# Autodesk Inventor assembly: Ensamblaje
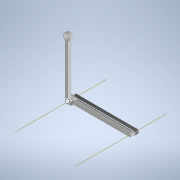
[picture p0: Inventor's stored thumbnail of the model, 180x180]
Saved by Autodesk Inventor 2021 (Build 250183000, 183)
## iProperties
Created: 2022-10-24
Part Number: Ensamblaje
Document SubType Name: Assembly
Designer: ivanm
Author: ivanm
## Documents named in this file (6)
- C:\Users\ivanm\OneDrive\Servomecanismos\Proyectos\Proyecto academico\Servomecanismo2R\INVENTOR\Ensamblaje.iam
- C:\Users\ivanm\OneDrive\Servomecanismos\Proyectos\Proyecto academico\Servomecanismo2R\INVENTOR\eslabon1.ipt
- C:\Users\ivanm\OneDrive\Servomecanismos\Proyectos\Proyecto academico\Servomecanismo2R\INVENTOR\eslabon2.ipt
- C:\Users\ivanm\OneDrive\Servomecanismos\Proyectos\Proyecto academico\Servomecanismo2R\INVENTOR\Eje1.ipt
- C:\Users\ivanm\OneDrive\Servomecanismos\Proyectos\Proyecto academico\Servomecanismo2R\INVENTOR\Ensamblaje\Design Accelerator\Transmisión de correas síncronas2.iam
- C:\Users\ivanm\OneDrive\Servomecanismos\Proyectos\Proyecto academico\Servomecanismo2R\INVENTOR\Ensamblaje\Design Accelerator\Rodamiento3.iam
## Components (5 placed, 5 different names)
1. eslabon1:1 — De rotación:1, Coincidencia:1, Nivelación:1
2. eslabon2:1 — De rotación:1, Rígido:1
3. Eje:1 — Rígido:1
4. Transmisión de correas síncronas:1 [sub-assembly]
5. Rodamiento:1 [sub-assembly] — Coincidencia:1, Nivelación:1
## Relationships (4: RevoluteJoint 1, WeldJoint 1, Mate 1, Flush 1)
- De rotación:1 [RevoluteJoint]: eslabon1:1 ↔ eslabon2:1
- Rígido:1 [WeldJoint]: eslabon2:1 ↔ Eje:1
- Coincidencia:1 [Mate]: eslabon1:1 ↔ Rodamiento:1
- Nivelación:1 [Flush]: eslabon1:1 ↔ Rodamiento:1
